# Autodesk Inventor assembly: 1_Body
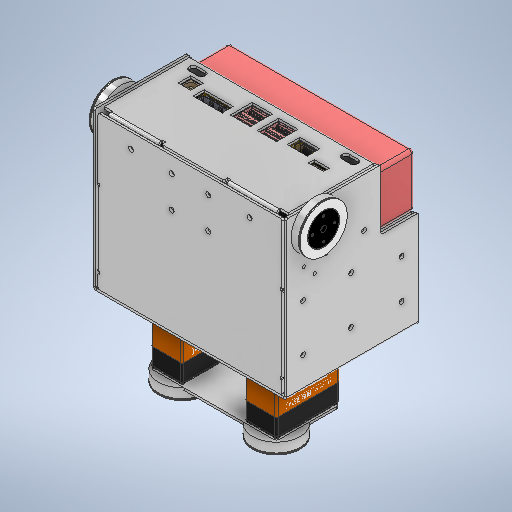
[picture p0: Inventor's stored thumbnail of the model, 512x512]
Saved by Autodesk Inventor 2025.2 (Build 292293000, 293)
## iProperties
Created: 2025-05-30
Part Number: 1_Body
Document SubType Name: Assembly
Designer: chris
Author: chris
## Documents named in this file (19)
- C:\Users\chris\Documents\Inventor\RHp_Humanoid_ver1\Assembly\1_Body.iam
- C:\Users\chris\Documents\Inventor\RHp_Humanoid_ver1\Part\Frame\Body\body_main_frame.ipt
- C:\Users\chris\Documents\Inventor\RHp_Humanoid_ver1\Part\Frame\Body\body_back_frame.ipt
- C:\Users\chris\Documents\Inventor\RHp_Humanoid_ver1\Part\Frame\Body\body_front_frame.ipt
- C:\Users\chris\Documents\Inventor\RHp_Humanoid_ver1\Part\Frame\Body\body_middle_frame.ipt
- C:\Users\chris\Documents\Inventor\RHp_Humanoid_ver1\Part\Frame\Body\body_motor_L_frame.ipt
- C:\Users\chris\Documents\Inventor\RHp_Humanoid_ver1\Part\Frame\Body\body_motor_R_frame.ipt
- C:\Users\chris\Documents\Inventor\RHp_Humanoid_ver1\Part\Frame\Body\body_top_frame.ipt
- C:\Users\chris\Documents\Inventor\RHp_Humanoid_ver1\Part\Other Parts\Servo_Driver.ipt
- C:\Users\chris\Documents\Inventor\RHp_Humanoid_ver1\Part\Other Parts\Battery_Pack.ipt
- C:\Users\chris\Documents\Inventor\RHp_Humanoid_ver1\Part\Other Parts\jetson_orin_super.ipt
- C:\Users\chris\Documents\Inventor\RHp_Humanoid_ver1\Part\HTD-45H, Horn\Horn\Top Horn.ipt
- C:\Users\chris\Documents\Inventor\RHp_Humanoid_ver1\Part\HTD-45H, Horn\HTD-45H\HTD-45H.iam
- C:\Users\chris\Documents\Inventor\RHp_Humanoid_ver1\Part\Frame\Body\body_bottom_frame.ipt
- C:\Users\chris\Documents\Inventor\RHp_Humanoid_ver1\Part\Other Parts\frame_motor_support_bottom_R.ipt
- C:\Users\chris\Documents\Inventor\RHp_Humanoid_ver1\Part\Other Parts\frame_motor_support_bottom_L.ipt
- C:\Users\chris\Documents\Inventor\RHp_Humanoid_ver1\Part\Other Parts\frame_motor_support_top_R.ipt
- C:\Users\chris\Documents\Inventor\RHp_Humanoid_ver1\Part\Other Parts\frame_motor_support_top_L.ipt
- C:\Users\chris\Documents\Inventor\RHp_Humanoid_ver1\Part\Bolt, Bearing, Nut, Washer\2030 Teflon Sheet.ipt
## Components (31 placed, 18 different names)
1. body_main_frame:1 — Mate:3, Flush:2, Mate:4, Mate:5, Flush:3, Flush:4, Mate:6, Flush:5, Mate:8, Mate:10, Mate:11, Flush:9, Flush:10, Mate:16, Mate:18, Flush:13, Mate:30, Flush:30, Flush:31, Mate:31, Mate:33, Mate:35, Mate:36, Flush:34, Flush:35, Mate:37, Mate:38, Mate:46, Mate:47, Mate:48, Mate:49, Mate:50, Mate:51
2. body_back_frame:1 — Mate:3, Flush:2, Mate:4, Mate:19
3. body_front_frame:1 — Mate:5, Flush:3, Flush:4, Flush:6, Mate:7, Flush:7, Mate:9, Flush:8
4. body_middle_frame:1 — Mate:6, Flush:5, Flush:6, Mate:17, Mate:28, Flush:29, Mate:29, Flush:32, Mate:32, Flush:33, Mate:34
5. body_motor_L_frame:1 — Mate:7, Flush:7, Mate:8
6. body_motor_R_frame:1 — Mate:9, Mate:10, Flush:8
7. body_top_frame:1 — Mate:11, Flush:9, Flush:10, Mate:20
8. Servo_Driver:1 — Mate:16, Mate:17, Mate:18
9. Battery_Pack:1 — Mate:19, Mate:20, Flush:13
10. jetson_orin_super:1 — Mate:28, Flush:29, Mate:29
11. Top Horn:1 — Rotational:1
12. Top Horn:2 — Rotational:2
13. HTD-45H:1 [sub-assembly] — Flush:32, Mate:31, Mate:32, Rotational:2
14. HTD-45H:2 [sub-assembly] — Flush:33, Mate:33, Mate:34, Rotational:1
15. HTD-45H:3 [sub-assembly] — Mate:35, Flush:34, Mate:38, Mate:39, Flush:36, Flush:37, Rotational:3
16. HTD-45H:4 [sub-assembly] — Mate:36, Flush:35, Mate:37, Rotational:4
17. body_bottom_frame:1 — Mate:39, Flush:36, Flush:37, Mate:40, Mate:41, Mate:42, Mate:43, Mate:44, Mate:45
18. frame_motor_support_bottom_R:1 — Mate:40, Mate:41, Mate:42, Insert:5
19. frame_motor_support_bottom_L:1 — Mate:43, Mate:44, Mate:45, Insert:7
20. frame_motor_support_top_R:1 — Mate:46, Mate:47, Mate:48, Insert:3
21. frame_motor_support_top_L:1 — Mate:49, Mate:50, Mate:51, Insert:1
22. Top Horn:3 — Rotational:4
23. Top Horn:4 — Rotational:3
24. 2030 Teflon Sheet:1 — Insert:1, Insert:2
25. 2030 Teflon Sheet:2 — Insert:2
26. 2030 Teflon Sheet:3 — Insert:3, Insert:4
27. 2030 Teflon Sheet:4 — Insert:4
28. 2030 Teflon Sheet:5 — Insert:5, Insert:6
29. 2030 Teflon Sheet:6 — Insert:6
30. 2030 Teflon Sheet:7 — Insert:7, Insert:8
31. 2030 Teflon Sheet:8 — Insert:8
## Relationships (69: Mate 38, Flush 19, Insert 8, RevoluteJoint 4)
- Mate:3: body_main_frame:1 ↔ body_back_frame:1
- Flush:2: body_main_frame:1 ↔ body_back_frame:1
- Mate:4: body_main_frame:1 ↔ body_back_frame:1
- Mate:5: body_main_frame:1 ↔ body_front_frame:1
- Flush:3 (1.5 mm): body_main_frame:1 ↔ body_front_frame:1
- Flush:4: body_main_frame:1 ↔ body_front_frame:1
- Mate:6: body_main_frame:1 ↔ body_middle_frame:1
- Flush:5 (1.5 mm): body_main_frame:1 ↔ body_middle_frame:1
- Flush:6 (-30 mm): body_front_frame:1 ↔ body_middle_frame:1
- Mate:7: body_front_frame:1 ↔ body_motor_L_frame:1
- Flush:7: body_front_frame:1 ↔ body_motor_L_frame:1
- Mate:8 (40 mm): body_main_frame:1 ↔ body_motor_L_frame:1
- Mate:9: body_front_frame:1 ↔ body_motor_R_frame:1
- Mate:10 (40 mm): body_main_frame:1 ↔ body_motor_R_frame:1
- Mate:11: body_main_frame:1 ↔ body_top_frame:1
- Flush:8: body_front_frame:1 ↔ body_motor_R_frame:1
- Flush:9: body_main_frame:1 ↔ body_top_frame:1
- Flush:10 (1.5 mm): body_main_frame:1 ↔ body_top_frame:1
- Mate:16 (10 mm): body_main_frame:1 ↔ Servo_Driver:1
- Mate:17: body_middle_frame:1 ↔ Servo_Driver:1
- Mate:18 (31 mm): body_main_frame:1 ↔ Servo_Driver:1
- Mate:19: body_back_frame:1 ↔ Battery_Pack:1
- Mate:20: body_top_frame:1 ↔ Battery_Pack:1
- Flush:13 (-2.5 mm): body_main_frame:1 ↔ Battery_Pack:1
- Mate:28: body_middle_frame:1 ↔ jetson_orin_super:1
- Flush:29 (6 mm): body_middle_frame:1 ↔ jetson_orin_super:1
- Mate:29 (7 mm): body_middle_frame:1 ↔ jetson_orin_super:1
- Mate:30: body_main_frame:1
- Flush:30: body_main_frame:1
- Flush:31: body_main_frame:1
- Flush:32: body_middle_frame:1 ↔ HTD-45H:1
- Mate:31: body_main_frame:1 ↔ HTD-45H:1
- Mate:32 (2 mm): body_middle_frame:1 ↔ HTD-45H:1
- Flush:33: body_middle_frame:1 ↔ HTD-45H:2
- Mate:33: body_main_frame:1 ↔ HTD-45H:2
- Mate:34 (2 mm): body_middle_frame:1 ↔ HTD-45H:2
- Rotational:1 [RevoluteJoint]: Top Horn:1 ↔ HTD-45H:2
- Rotational:2 [RevoluteJoint]: Top Horn:2 ↔ HTD-45H:1
- Mate:35: body_main_frame:1 ↔ HTD-45H:3
- Mate:36: body_main_frame:1 ↔ HTD-45H:4
- Flush:34 (15 mm): body_main_frame:1 ↔ HTD-45H:3
- Flush:35 (15 mm): body_main_frame:1 ↔ HTD-45H:4
- Mate:37 (20 mm): body_main_frame:1 ↔ HTD-45H:4
- Mate:38 (20 mm): body_main_frame:1 ↔ HTD-45H:3
- Mate:39: HTD-45H:3 ↔ body_bottom_frame:1
- Flush:36: HTD-45H:3 ↔ body_bottom_frame:1
- Flush:37: HTD-45H:3 ↔ body_bottom_frame:1
- Mate:40: body_bottom_frame:1 ↔ frame_motor_support_bottom_R:1
- Mate:41: body_bottom_frame:1 ↔ frame_motor_support_bottom_R:1
- Mate:42: body_bottom_frame:1 ↔ frame_motor_support_bottom_R:1
- Mate:43: body_bottom_frame:1 ↔ frame_motor_support_bottom_L:1
- Mate:44: body_bottom_frame:1 ↔ frame_motor_support_bottom_L:1
- Mate:45: body_bottom_frame:1 ↔ frame_motor_support_bottom_L:1
- Mate:46: body_main_frame:1 ↔ frame_motor_support_top_R:1
- Mate:47: body_main_frame:1 ↔ frame_motor_support_top_R:1
- Mate:48: body_main_frame:1 ↔ frame_motor_support_top_R:1
- Mate:49: body_main_frame:1 ↔ frame_motor_support_top_L:1
- Mate:50: body_main_frame:1 ↔ frame_motor_support_top_L:1
- Mate:51: body_main_frame:1 ↔ frame_motor_support_top_L:1
- Rotational:3 [RevoluteJoint]: HTD-45H:3 ↔ Top Horn:4
- Rotational:4 [RevoluteJoint]: HTD-45H:4 ↔ Top Horn:3
- Insert:1: frame_motor_support_top_L:1 ↔ 2030 Teflon Sheet:1
- Insert:2 (0.07 mm): 2030 Teflon Sheet:1 ↔ 2030 Teflon Sheet:2
- Insert:3: frame_motor_support_top_R:1 ↔ 2030 Teflon Sheet:3
- Insert:4 (0.07 mm): 2030 Teflon Sheet:3 ↔ 2030 Teflon Sheet:4
- Insert:5: frame_motor_support_bottom_R:1 ↔ 2030 Teflon Sheet:5
- Insert:6 (0.07 mm): 2030 Teflon Sheet:5 ↔ 2030 Teflon Sheet:6
- Insert:7: frame_motor_support_bottom_L:1 ↔ 2030 Teflon Sheet:7
- Insert:8 (0.07 mm): 2030 Teflon Sheet:7 ↔ 2030 Teflon Sheet:8
